# Autodesk Inventor assembly: linear slide
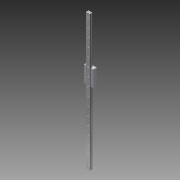
[picture p0: Inventor's stored thumbnail of the model, 180x180]
Saved by Autodesk Inventor 2015 (Build 190159000, 159)
## iProperties
Created: 2015-01-29
Part Number: linear slide
Document SubType Name: Assembly
Designer: Joseph
Author: Joseph
## Documents named in this file (3)
- Z:\CloudStation\3d models\Kossel\linear slide.iam
- Z:\CloudStation\3d models\Kossel\slide rail.ipt
- Z:\CloudStation\3d models\Kossel\slide.ipt
## Components (2 placed, 2 different names)
1. slide rail:1 — Slider:1
2. slide:1 — Slider:1
## Relationships (1: TranslationJoint 1)
- Slider:1 [TranslationJoint]: slide rail:1 ↔ slide:1
